# Autodesk Inventor assembly: Assemblything
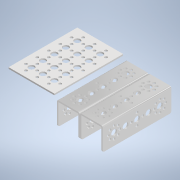
[picture p0: Inventor's stored thumbnail of the model, 180x180]
Saved by Autodesk Inventor 2020.1 (Build 241239000, 239)
## iProperties
Created: 2019-12-06
Part Number: Assemblything
Document SubType Name: Assembly
Designer: tbloo
Author: tbloo
## Documents named in this file (3)
- C:\Users\tbloo\Documents\GitHub\AO_Robotics\CAD\Projects\Timothy Bloot\Assemblything.iam
- C:\Users\tbloo\Documents\GitHub\AO_Robotics\CAD\Parts Kits\FTC Tetrix KOP Organized (7-24-19)\Frame Hardware\Tetrix_39066.ipt
- C:\Users\tbloo\Documents\GitHub\AO_Robotics\CAD\Projects\Timothy Bloot\Tango\Part4.ipt
## Components (3 placed, 2 different names)
1. Tetrix_39066:1 — Flush:1, Flush:2, Mate:1, Flush:3
2. Tetrix_39066:2 — Flush:1, Flush:2, Mate:1
3. Part4:1 — Flush:3
## Relationships (4: Flush 3, Mate 1)
- Flush:1: Tetrix_39066:1 ↔ Tetrix_39066:2
- Flush:2: Tetrix_39066:1 ↔ Tetrix_39066:2
- Mate:1: Tetrix_39066:1 ↔ Tetrix_39066:2
- Flush:3: Tetrix_39066:1 ↔ Part4:1
